# Autodesk Inventor assembly: ISSOKU_Ballscrew_D12x160_05_590104-13
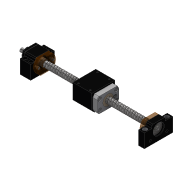
[picture p0: Inventor's stored thumbnail of the model, 180x180]
Saved by Autodesk Inventor 2016 (Build 200138000, 138)
## iProperties
Created: 2015-07-27
Part Number: ISSOKU_Ballscrew_D12x160_05_590104-13
Document SubType Name: Assembly
## Documents named in this file (16)
- C:\Dropbox\Inventor\Projects\Portalfraese_V2_Z-Axis\ISSOKU_Ballscrew_D12x160_05_590104-13.iam
- C:\Dropbox\Inventor\Projects\Portalfraese_V2_Z-Axis\7000ADFMP5.ipt
- C:\Dropbox\Inventor\Projects\Portalfraese_V2_Z-Axis\Ballnut_Support.ipt
- C:\Dropbox\Inventor\Projects\Portalfraese_V2_Z-Axis\Endpuffer.ipt
- C:\Dropbox\Inventor\Projects\Portalfraese_V2_Z-Axis\Festlager Deckel.ipt
- C:\Dropbox\Inventor\Projects\Portalfraese_V2_Z-Axis\ISSOKU_Ballnut_05_590104-13.ipt
- C:\Dropbox\Inventor\Projects\Portalfraese_V2_Z-Axis\Lagerbock_Festlager.ipt
- C:\Dropbox\Inventor\Projects\Portalfraese_V2_Z-Axis\Lagerbock_Loslager.ipt
- C:\Dropbox\Inventor\Projects\Portalfraese_V2_Z-Axis\Spindel.ipt
- C:\Dropbox\Inventor\Projects\Portalfraese_V2_Z-Axis\Wellenmutter.ipt
- C:\Dropbox\Inventor\Projects\Portalfraese_V2_Z-Axis\608-2Z.ipt
- C:\Dropbox\Inventor\Projects\Portalfraese_V2_Z-Axis\Sicherungsring_DIN471_D8.ipt
- C:\Dropbox\Inventor\Projects\001_EK-Teile\Zyl-Schr_ISO 4762 - M3 x 6_St-Vzkt.ipt
- C:\Dropbox\Inventor\Projects\001_EK-Teile\Zyl-Schr_ISO 4762 - M3 x 8_St-Vzkt.ipt
- C:\Dropbox\Inventor\Projects\001_EK-Teile\Zyl-Schr_ISO 4762 - M4 x 10_St-Vzkt.ipt
- C:\Dropbox\Inventor\Projects\001_EK-Teile\Gewindestift_ISO 4026 - M4 x 5_St-B.ipt
## Components (25 placed, 14 different names)
1. 7000ADFMP5:1 — Insert:2, Insert:3, Insert:4, Insert:5
2. Ballnut_Support:2 — Mate:3, Mate:4, Mate:5, Mate:9, Angle:1
3. Endpuffer:3 — Insert:1, Mate:9, Insert:13, Insert:14
4. Festlager Deckel:4 — Insert:3, Mate:1, Insert:9, Insert:10, Insert:11, Insert:12
5. ISSOKU_Ballnut_05_590104-13:5 — Mate:2, Mate:3, Mate:4, Mate:5, Insert:17, Insert:18, Insert:19, Insert:20
6. Lagerbock_Loslager:6 — Insert:1, Insert:2, Mate:1, Flush:1, Angle:1
7. Lagerbock_Loslager:7 — Mate:6, Insert:8, Mate:7, Flush:1
8. Spindel:8 — Insert:4, Mate:2, Insert:6, Insert:7, Tangent:1
9. Wellenmutter:9 — Insert:5, Mate:10
10. Endpuffer:10 — Insert:8, Mate:7, Mate:8, Insert:15, Insert:16
11. 608-2Z:11 — Insert:7, Mate:6, Mate:8
12. Sicherungsring_DIN471_D8:12 — Insert:6
13. ISO 4762 - M3 x 6:13 — Insert:12
14. ISO 4762 - M3 x 8:14 — Insert:14
15. ISO 4762 - M4 x 10:15 — Insert:17
16. ISO 4762 - M3 x 6:16 — Insert:9
17. ISO 4762 - M3 x 6:17 — Insert:10
18. ISO 4762 - M3 x 6:18 — Insert:11
19. ISO 4762 - M3 x 8:19 — Insert:16
20. ISO 4762 - M3 x 8:20 — Insert:15
21. ISO 4762 - M3 x 8:21 — Insert:13
22. ISO 4762 - M4 x 10:22 — Insert:18
23. ISO 4762 - M4 x 10:23 — Insert:20
24. ISO 4762 - M4 x 10:24 — Insert:19
25. ISO 4026 - M4 x 5:25 — Mate:10, Tangent:1
## Relationships (33: Insert 20, Mate 10, Flush 1, Angle 1, Tangent 1)
- Insert:1: Endpuffer:3 ↔ Lagerbock_Loslager:6
- Insert:2: 7000ADFMP5:1 ↔ Lagerbock_Loslager:6
- Insert:3: 7000ADFMP5:1 ↔ Festlager Deckel:4
- Mate:1: Festlager Deckel:4 ↔ Lagerbock_Loslager:6
- Insert:4: 7000ADFMP5:1 ↔ Spindel:8
- Insert:5: 7000ADFMP5:1 ↔ Wellenmutter:9
- Mate:2: ISSOKU_Ballnut_05_590104-13:5 ↔ Spindel:8
- Mate:3: Ballnut_Support:2 ↔ ISSOKU_Ballnut_05_590104-13:5
- Mate:4: Ballnut_Support:2 ↔ ISSOKU_Ballnut_05_590104-13:5
- Mate:5: Ballnut_Support:2 ↔ ISSOKU_Ballnut_05_590104-13:5
- Insert:6: Spindel:8 ↔ Sicherungsring_DIN471_D8:12
- Insert:7: Spindel:8 ↔ 608-2Z:11
- Mate:6: Lagerbock_Loslager:7 ↔ 608-2Z:11
- Insert:8: Lagerbock_Loslager:7 ↔ Endpuffer:10
- Mate:7: Lagerbock_Loslager:7 ↔ Endpuffer:10
- Mate:8: Endpuffer:10 ↔ 608-2Z:11
- Flush:1: Lagerbock_Loslager:6 ↔ Lagerbock_Loslager:7
- Mate:9: Ballnut_Support:2 ↔ Endpuffer:3
- Angle:1 (180 deg): Ballnut_Support:2 ↔ Lagerbock_Loslager:6
- Insert:9: Festlager Deckel:4 ↔ ISO 4762 - M3 x 6:16
- Insert:10: Festlager Deckel:4 ↔ ISO 4762 - M3 x 6:17
- Insert:11: Festlager Deckel:4 ↔ ISO 4762 - M3 x 6:18
- Insert:12: Festlager Deckel:4 ↔ ISO 4762 - M3 x 6:13
- Insert:13: Endpuffer:3 ↔ ISO 4762 - M3 x 8:21
- Insert:14: Endpuffer:3 ↔ ISO 4762 - M3 x 8:14
- Insert:15: Endpuffer:10 ↔ ISO 4762 - M3 x 8:20
- Insert:16: Endpuffer:10 ↔ ISO 4762 - M3 x 8:19
- Insert:17: ISSOKU_Ballnut_05_590104-13:5 ↔ ISO 4762 - M4 x 10:15
- Insert:18: ISSOKU_Ballnut_05_590104-13:5 ↔ ISO 4762 - M4 x 10:22
- Insert:19: ISSOKU_Ballnut_05_590104-13:5 ↔ ISO 4762 - M4 x 10:24
- Insert:20: ISSOKU_Ballnut_05_590104-13:5 ↔ ISO 4762 - M4 x 10:23
- Mate:10: Wellenmutter:9 ↔ ISO 4026 - M4 x 5:25
- Tangent:1: Spindel:8 ↔ ISO 4026 - M4 x 5:25
